# Autodesk Inventor assembly: Assembly positive and negative emboss
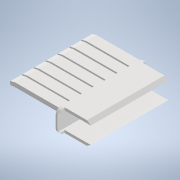
[picture p0: Inventor's stored thumbnail of the model, 180x180]
Saved by Autodesk Inventor 2020.2 (Build 242310000, 310)
## iProperties
Created: 2020-05-05
Part Number: Assembly positive and negative emboss
Document SubType Name: Assembly
Designer: Amaan Khalid
Author: Amaan Khalid
## Documents named in this file (3)
- C:\Users\Amaan Khalid\Desktop\my projects\my jumper cablehodler\Assembly positive and negative emboss.iam
- C:\Users\Amaan Khalid\Desktop\my projects\my jumper cablehodler\the whole thing.ipt
- C:\Users\Amaan Khalid\Desktop\my projects\my jumper cablehodler\hook thing.ipt
## Components (8 placed, 2 different names)
1. the whole thing:1 — Mate:1, Flush:1, Mate:2, Flush:2, Mate:3, Flush:3, Mate:4, Flush:4, Mate:5, Flush:5, Mate:6, Flush:6, Mate:7, Flush:7
2. hook thing:3 — Mate:1, Flush:1
3. hook thing:4 — Mate:2, Flush:2
4. hook thing:5 — Mate:3, Flush:3
5. hook thing:6 — Mate:4, Flush:4
6. hook thing:7 — Mate:5, Flush:5
7. hook thing:8 — Mate:6, Flush:6
8. hook thing:9 — Mate:7, Flush:7
## Relationships (14: Mate 7, Flush 7)
- Mate:1: the whole thing:1 ↔ hook thing:3
- Flush:1: the whole thing:1 ↔ hook thing:3
- Mate:2: the whole thing:1 ↔ hook thing:4
- Flush:2: the whole thing:1 ↔ hook thing:4
- Mate:3: the whole thing:1 ↔ hook thing:5
- Flush:3: the whole thing:1 ↔ hook thing:5
- Mate:4: the whole thing:1 ↔ hook thing:6
- Flush:4: the whole thing:1 ↔ hook thing:6
- Mate:5: the whole thing:1 ↔ hook thing:7
- Flush:5: the whole thing:1 ↔ hook thing:7
- Mate:6: the whole thing:1 ↔ hook thing:8
- Flush:6: the whole thing:1 ↔ hook thing:8
- Mate:7: the whole thing:1 ↔ hook thing:9
- Flush:7: the whole thing:1 ↔ hook thing:9
